# Autodesk Inventor assembly: A_MiniDrone
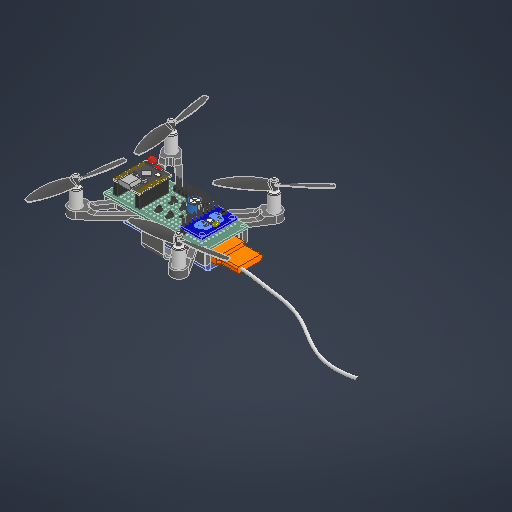
[picture p0: Inventor's stored thumbnail of the model, 512x512]
Saved by Autodesk Inventor 2026 (Build 300175000, 175)
## iProperties
Created: 2025-08-01
Part Number: A_MiniDrone
Document SubType Name: Assembly
Designer: FAL
Author: FAL
## Documents named in this file (10)
- C:\Users\FAL\Projekte\local\MiniDrone\Hardware\CAD\V2\A_MiniDrone.iam
- C:\Users\FAL\Projekte\local\MiniDrone\Hardware\CAD\V2\P_DroneCase.ipt
- C:\Users\FAL\Projekte\local\MiniDrone\Hardware\CAD\V2\extern\ESP32-C3 supermini v5\ESP32-C3 supermini v5\ESP32-C3 supermini v5.iam
- C:\Users\FAL\Projekte\local\MiniDrone\Hardware\CAD\V2\P_Akku_1S.ipt
- C:\Users\FAL\Projekte\local\MiniDrone\Hardware\CAD\V2\P_Motor.ipt
- C:\Users\FAL\Projekte\local\MiniDrone\Hardware\CAD\V2\P_Prop.ipt
- C:\Users\FAL\Projekte\local\MiniDrone\Hardware\CAD\V2\P_R6DSM.ipt
- C:\Users\FAL\Projekte\local\MiniDrone\Hardware\Platine\MiniDroneFlightcontroller\MiniDroneFlightcontroller\MiniDroneFlightcontroller\MiniDroneFlightcontroller.iam
- C:\Users\FAL\Projekte\local\MiniDrone\Hardware\CAD\V2\extern\MPU9250\MPU-9250.iam
- C:\Users\FAL\Projekte\local\MiniDrone\Hardware\CAD\V2\P_Halter.ipt
## Components (15 placed, 9 different names)
1. P_DroneCase:1 — Passend:1, Passend:2, Fluchtend:1, Passend:3, Passend:4, Passend:5, Passend:6, Fluchtend:9, Passend:19, Fluchtend:21, Fluchtend:24, Passend:22
2. ESP32-C3 supermini v5:1 [sub-assembly] — Fluchtend:22, Passend:20
3. P_Akku_1S:1
4. P_Motor:1 — Passend:3, Fluchtend:3, Passend:8
5. P_Motor:2 — Passend:4, Fluchtend:3, Fluchtend:4, Fluchtend:5, Passend:7
6. P_Motor:3 — Passend:5, Fluchtend:5, Passend:9, Passend:11, Fluchtend:24
7. P_Motor:4 — Passend:6, Fluchtend:4, Passend:10
8. P_Prop:1 — Passend:7, Fluchtend:6
9. P_Prop:2 — Passend:8, Fluchtend:6, Fluchtend:7
10. P_Prop:3 — Passend:10, Fluchtend:7, Fluchtend:8
11. P_Prop:4 — Passend:9, Fluchtend:8, Passend:11
12. P_R6DSM:1
13. MiniDroneFlightcontroller:1 [sub-assembly] — Fluchtend:9, Passend:19, Fluchtend:21, Fluchtend:22, Passend:20, Passend:21, Fluchtend:23
14. MPU-9250:1 [sub-assembly] — Passend:21, Fluchtend:23
15. P_Halter:1 — Passend:22
## Relationships (27: Mate 15, Flush 12)
- Passend:1 [Mate]: P_DroneCase:1
- Passend:2 [Mate]: P_DroneCase:1
- Fluchtend:1 [Flush]: P_DroneCase:1
- Passend:3 [Mate]: P_DroneCase:1 ↔ P_Motor:1
- Passend:4 [Mate]: P_DroneCase:1 ↔ P_Motor:2
- Passend:5 [Mate]: P_DroneCase:1 ↔ P_Motor:3
- Passend:6 [Mate]: P_DroneCase:1 ↔ P_Motor:4
- Fluchtend:3 [Flush]: P_Motor:1 ↔ P_Motor:2
- Fluchtend:4 [Flush]: P_Motor:2 ↔ P_Motor:4
- Fluchtend:5 [Flush]: P_Motor:2 ↔ P_Motor:3
- Passend:7 [Mate]: P_Motor:2 ↔ P_Prop:1
- Passend:8 [Mate]: P_Motor:1 ↔ P_Prop:2
- Passend:9 [Mate]: P_Motor:3 ↔ P_Prop:4
- Passend:10 [Mate]: P_Motor:4 ↔ P_Prop:3
- Fluchtend:6 [Flush]: P_Prop:1 ↔ P_Prop:2
- Fluchtend:7 [Flush]: P_Prop:2 ↔ P_Prop:3
- Fluchtend:8 [Flush]: P_Prop:3 ↔ P_Prop:4
- Passend:11 [Mate] (1 mm): P_Motor:3 ↔ P_Prop:4
- Fluchtend:9 [Flush]: P_DroneCase:1 ↔ MiniDroneFlightcontroller:1
- Passend:19 [Mate]: P_DroneCase:1 ↔ MiniDroneFlightcontroller:1
- Fluchtend:21 [Flush]: P_DroneCase:1 ↔ MiniDroneFlightcontroller:1
- Fluchtend:22 [Flush]: ESP32-C3 supermini v5:1 ↔ MiniDroneFlightcontroller:1
- Passend:20 [Mate]: ESP32-C3 supermini v5:1 ↔ MiniDroneFlightcontroller:1
- Passend:21 [Mate]: MiniDroneFlightcontroller:1 ↔ MPU-9250:1
- Fluchtend:23 [Flush]: MiniDroneFlightcontroller:1 ↔ MPU-9250:1
- Fluchtend:24 [Flush]: P_DroneCase:1 ↔ P_Motor:3
- Passend:22 [Mate]: P_DroneCase:1 ↔ P_Halter:1
